# Autodesk Inventor assembly: Передача с помощью зубчатых ремней
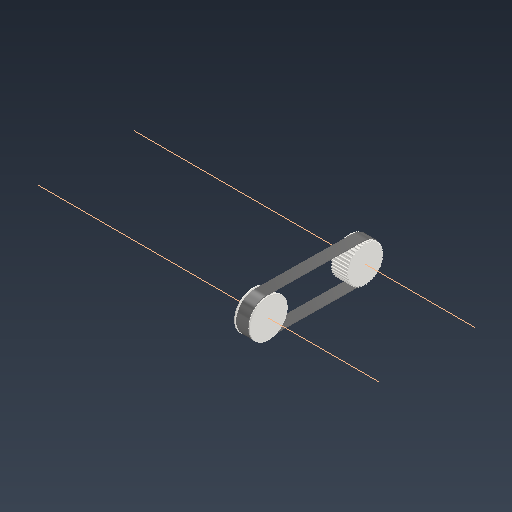
[picture p0: Inventor's stored thumbnail of the model, 512x512]
Saved by Autodesk Inventor 2025 (Build 290162000, 162)
## iProperties
ClientObjectVersion: 1
Created: 2025-09-22
Part Number: Передача с помощью зубчатых ремней
Document SubType Name: Assembly
Designer: GameHD
Author: GameHD
## Documents named in this file (4)
- C:\Users\GameHD\Desktop\Phantom 16950\цепь\Мастер проектирования\Передача с помощью зубчатых ремней1.iam
- C:\Users\GameHD\Desktop\Phantom 16950\цепь\Мастер проектирования\Зубчатый ремень1.ipt
- C:\Users\GameHD\Desktop\Phantom 16950\цепь\Мастер проектирования\Синхронный шкив11.ipt
- C:\Users\GameHD\Desktop\Phantom 16950\цепь\Мастер проектирования\Синхронный шкив21.ipt
## Components (3 placed, 3 different names)
1. Зубчатый ремень:1 — Заподлицо:1, Совмещение:1, Совмещение:2, Заподлицо:2, Совмещение:3, Совмещение:4
2. Синхронный шкив1:1 — Заподлицо:1, Совмещение:1, Совмещение:2, ЗубчПер:1
3. Синхронный шкив2:1 — Заподлицо:2, Совмещение:3, ЗубчПер:1, Совмещение:4
## Relationships (7: Mate 4, Flush 2, RelateRotation 1)
- Заподлицо:1 [Flush]: Зубчатый ремень:1 ↔ Синхронный шкив1:1
- Совмещение:1 [Mate]: Зубчатый ремень:1 ↔ Синхронный шкив1:1
- Совмещение:2 [Mate]: Зубчатый ремень:1 ↔ Синхронный шкив1:1
- Заподлицо:2 [Flush]: Зубчатый ремень:1 ↔ Синхронный шкив2:1
- Совмещение:3 [Mate]: Зубчатый ремень:1 ↔ Синхронный шкив2:1
- ЗубчПер:1 [RelateRotation] (1 ul): Синхронный шкив1:1 ↔ Синхронный шкив2:1
- Совмещение:4 [Mate]: Зубчатый ремень:1 ↔ Синхронный шкив2:1
